# Autodesk Inventor assembly: intake part on end of six bar_MIR
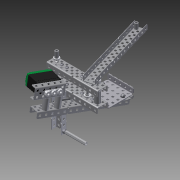
[picture p0: Inventor's stored thumbnail of the model, 180x180]
Saved by Autodesk Inventor 2014 SP1 (Build 180222100, 222)
## iProperties
Created: 2014-02-27
Part Number: intake part on end of six bar_MIR
Document SubType Name: Assembly
Designer: Ryan
Author: Ryan
## Documents named in this file (22)
- C:\Users\Ryan\Desktop\sw\toss up 4th robot\intake\intake part on end of six bar_MIR.iam
- C:\Users\Ryan\Desktop\sw\lib\Aperture VEX CAD Library\Metal\C Channel\2 x 10.ipt
- C:\Users\Ryan\Desktop\sw\lib\Aperture VEX CAD Library\Metal\C Channel\2 x 7.ipt
- C:\Users\Ryan\Desktop\sw\lib\Aperture VEX CAD Library\Bearing Blocks\Bearing Block.ipt
- C:\Users\Ryan\Desktop\sw\lib\Aperture VEX CAD Library\Metal\C Channel\5 x 5.ipt
- C:\Users\Ryan\Desktop\sw\lib\Aperture VEX CAD Library\Metal\vex hinge\hinge.iam
- C:\Users\Ryan\Desktop\sw\lib\Aperture VEX CAD Library\Spacers\SPACER-0500-0125.ipt
- C:\Users\Ryan\Desktop\sw\lib\Aperture VEX CAD Library\Spacers\SPACER-0500-0500.ipt
- C:\Users\Ryan\Desktop\sw\lib\Aperture VEX CAD Library\Spacers\SPACER-0500-0250.ipt
- C:\Users\Ryan\Desktop\sw\lib\Aperture VEX CAD Library\Metal\C Channel\2 x 15.ipt
- C:\Users\Ryan\Desktop\sw\toss up 4th robot\intake\4 hole long poly.ipt
- C:\Users\Ryan\Desktop\sw\lib\Aperture VEX CAD Library\Metal\C Channel\2 x 5.ipt
- C:\Users\Ryan\Desktop\sw\lib\Aperture VEX CAD Library\Motors\2-Wire Motor 393-Without Wire.iam
- C:\Users\Ryan\Desktop\sw\lib\Aperture VEX CAD Library\Standoffs\BEAM-2000.ipt
- C:\Users\Ryan\Desktop\sw\lib\Aperture VEX CAD Library\Hardware\8-32\8-32 nylock.ipt
- C:\Users\Ryan\Desktop\sw\lib\Aperture VEX CAD Library\Spacers\thin\SPACER-0320-0500.ipt
- C:\Users\Ryan\Desktop\sw\lib\Aperture VEX CAD Library\Hardware\8-32\8-32_.500.ipt
- C:\Users\Ryan\Desktop\sw\lib\Aperture VEX CAD Library\Hardware\8-32\8-32_.375.ipt
- C:\Users\Ryan\Desktop\sw\lib\Aperture VEX CAD Library\Hardware\8-32\8-32_.875.ipt
- C:\Users\Ryan\Desktop\sw\lib\Aperture VEX CAD Library\Hardware\8-32\8-32_1.750.ipt
- C:\Users\Ryan\Desktop\sw\lib\Aperture VEX CAD Library\Hardware\8-32\8-32 nylock_MIR7.ipt
- C:\Users\Ryan\Desktop\sw\lib\Aperture VEX CAD Library\Spacers\thin\SPACER-0320-00625.ipt
## Components (77 placed, 21 different names)
1. 2 x 10:1 — Flush:2, Flush:1, Flush:4, Flush:3, Mate:1, Mate:3, Mate:2, Mate:7, Mate:5, Mate:10, Mate:9, Mate:8, Mate:6, Flush:6, Flush:5, Mate:11, Mate:20, Mate:148
2. 2 x 10:2 — Flush:2, Flush:1, Mate:19, Mate:18, Mate:71, Mate:70, Mate:69, Mate:72, Mate:75, Mate:88, Mate:87, Mate:86, Mate:96, Mate:95, Mate:99, Mate:100, Mate:129, Mate:132, Mate:145, Mate:154
3. 2 x 7:1 — Flush:4, Flush:3, Mate:1, Mate:80, Mate:79, Mate:78
4. Bearing Block:1 — Mate:3, Mate:2, Mate:7, Mate:5, Mate:77, Mate:76, Mate:136
5. Bearing Block:2 — Mate:10, Mate:9, Mate:8, Mate:6, Mate:74, Mate:73, Mate:134
6. 5 x 5:1 — Flush:6, Flush:5, Mate:11, Flush:8, Flush:7, Mate:12, Mate:23, Mate:22, Mate:21, Mate:26, Mate:25, Mate:24, Mate:122, Mate:124
7. hinge:1 [sub-assembly] — Flush:8, Flush:7, Mate:12, Mate:29, Mate:28, Mate:27, Mate:126
8. SPACER-0500-0125:1 — Mate:15, Mate:16, Mate:146, Mate:147
9. SPACER-0500-0500:1 — Mate:20, Mate:15, Mate:14, Mate:13
10. SPACER-0500-0500:2 — Mate:19, Mate:18, Mate:16, Mate:14, Mate:13
11. SPACER-0500-0125:2 — Mate:23, Mate:22, Mate:21, Mate:118, Mate:117
12. SPACER-0500-0125:3 — Mate:26, Mate:25, Mate:24, Mate:120, Mate:119, Mate:121
13. SPACER-0500-0250:1 — Mate:29, Mate:28, Mate:27, Mate:30, Mate:35
14. 2 x 15:1 — Mate:30, Mate:33, Mate:32, Mate:31, Mate:40, Mate:39, Mate:38, Mate:37, Mate:36, Mate:46, Mate:45, Mate:44, Mate:53, Mate:52, Mate:51, Mate:110, Mate:112, Mate:142, Mate:144, Mate:139, Mate:141, Mate:142
15. Bearing Block:3 — Mate:35, Mate:33, Mate:32, Mate:31, Mate:109, Mate:111, Mate:114, Mate:115, Mate:125, Mate:128
16. SPACER-0500-0250:2 — Mate:40, Mate:39, Flush:9, Mate:43, Mate:137
17. SPACER-0500-0250:3 — Flush:9, Mate:38, Mate:37, Mate:36, Mate:42, Mate:41, Mate:139, Mate:141
18. 4 hole long poly:1 — Mate:43, Mate:42, Mate:41, Mate:138, Mate:140
19. SPACER-0500-0500:3 — Mate:46, Mate:45, Mate:44, Mate:48, Mate:47
20. SPACER-0500-0500:4 — Mate:48, Mate:47, Mate:57, Mate:54, Mate:140
21. SPACER-0500-0500:5 — Mate:53, Mate:52, Mate:51, Mate:50, Mate:49
22. SPACER-0500-0500:6 — Mate:50, Mate:49, Mate:56, Mate:55
23. 2 x 5:1 — Mate:57, Mate:56, Mate:55, Mate:54, Mate:61, Mate:60, Mate:59, Mate:58, Mate:62, Mate:140
24. Bearing Block:4 — Mate:61, Mate:60, Mate:59, Mate:58, Mate:64, Mate:63
25. 2-Wire Motor 393-Without Wire:1 [sub-assembly] — Mate:64, Mate:63, Mate:62
26. 2 x 15:2 — Mate:68, Mate:67, Mate:66, Mate:85, Mate:84, Mate:83
27. SPACER-0500-0125:4 — Mate:71, Mate:70, Mate:69, Mate:68, Mate:67, Mate:66, Mate:152, Mate:153
28. Bearing Block:5 — Mate:74, Mate:73, Mate:72, Mate:90, Mate:89, Mate:94, Mate:93, Mate:101, Mate:104, Mate:130
29. Bearing Block:6 — Mate:77, Mate:76, Mate:75, Mate:92, Mate:91, Mate:98, Mate:97, Mate:105, Mate:108, Mate:131
30. BEAM-2000:1 — Mate:82, Mate:81
31. 8-32 nylock:1 — Mate:82, Mate:81, Mate:80, Mate:79, Mate:78
32. SPACER-0320-0500:1 — Mate:85, Mate:84, Mate:83
33. SPACER-0320-0500:2 — Mate:88, Mate:87, Mate:86, Mate:155, Mate:156, Mate:157
34. SPACER-0500-0250:4 — Mate:90, Mate:89
35. SPACER-0500-0250:5 — Mate:92, Mate:91
36. 8-32_.500:5 — Mate:110, Mate:109, Mate:113
37. 8-32_.500:6 — Mate:112, Mate:111, Mate:116, Mate:139
38. 8-32 nylock:6 — Mate:114, Mate:113
39. 8-32 nylock:7 — Mate:116, Mate:115
40. 8-32_.375:1 — Mate:118, Mate:117, Mate:123
41. 8-32_.375:2 — Mate:120, Mate:119
42. 8-32 nylock:8 — Mate:122, Mate:121
43. 8-32 nylock:9 — Mate:124, Mate:123
44. 8-32_.875:1 — Mate:126, Mate:125, Mate:127
45. 8-32 nylock:10 — Mate:128, Mate:127
46. 8-32_1.750:1 — Mate:130, Mate:129, Mate:133
47. 8-32_1.750:2 — Mate:132, Mate:131, Mate:135, Mate:149, Mate:151
48. 8-32 nylock_MIR7:1 — Mate:134, Mate:133
49. 8-32 nylock:11 — Mate:136, Mate:135
50. 8-32_.500:7 — Mate:138, Mate:137, Mate:141
51. 8-32_.500:8 — Mate:140, Mate:139, Mate:143
52. 8-32 nylock:12 — Mate:142, Mate:141
53. 8-32 nylock:13 — Mate:144, Mate:143, Mate:142
54. SPACER-0500-0125:5 — Mate:143, Mate:144, Mate:146, Mate:147
55. SPACER-0500-0125:6 — Mate:143, Mate:144, Mate:145
56. SPACER-0500-0125:7 — Mate:148, Mate:149, Mate:150
57. SPACER-0320-00625:1 — Mate:150, Mate:151
58. SPACER-0500-0125:8 — Mate:152, Mate:153, Mate:158, Mate:159
59. SPACER-0500-0125:9 — Mate:154, Mate:155
60. SPACER-0320-00625:2 — Mate:156, Mate:157
61. SPACER-0320-00625:3 — Mate:158, Mate:159
62. 8-32_.500:3 — Mate:99, Mate:98, Mate:107
63. 8-32_.500:4 — Mate:100, Mate:97, Mate:106
64. 8-32_.500:1 — Mate:96, Mate:94, Mate:103
65. 8-32_.500:2 — Mate:95, Mate:93, Mate:102
66. 8-32 nylock:5 — Mate:108, Mate:107
67. 8-32 nylock:4 — Mate:106, Mate:105
68. 8-32 nylock:2 — Mate:102, Mate:101
69. 8-32 nylock:3 — Mate:104, Mate:103
70. 8-32_.500:9
71. 8-32_.500:10
72. 8-32_.500:11
73. 8-32_.500:12
74. 8-32 nylock:14
75. 8-32 nylock:15
76. 8-32 nylock:16
77. 8-32 nylock:17
## Component patterns: (2 elements, first: 8-32_.500:3 + 8-32_.500:4 + 8-32_.500:1 + 8-32_.500:2 + 8-32 nylock:5 + 8-32 nylock:4 + 8-32 nylock:2 + 8-32 nylock:3)
## Relationships (170: Mate 157, Flush 13)
- Flush:2: 2 x 10:1 ↔ 2 x 10:2
- Flush:1: 2 x 10:1 ↔ 2 x 10:2
- Flush:4: 2 x 10:1 ↔ 2 x 7:1
- Flush:3: 2 x 10:1 ↔ 2 x 7:1
- Mate:1: 2 x 10:1 ↔ 2 x 7:1
- Mate:3 (2.3114 mm): 2 x 10:1 ↔ Bearing Block:1
- Mate:2: 2 x 10:1 ↔ Bearing Block:1
- Mate:7 (2.3114 mm): 2 x 10:1 ↔ Bearing Block:1
- Mate:5 (2.3114 mm): 2 x 10:1 ↔ Bearing Block:1
- Mate:10 (2.3114 mm): 2 x 10:1 ↔ Bearing Block:2
- Mate:9 (2.3114 mm): 2 x 10:1 ↔ Bearing Block:2
- Mate:8 (2.3114 mm): 2 x 10:1 ↔ Bearing Block:2
- Mate:6: 2 x 10:1 ↔ Bearing Block:2
- Flush:6: 2 x 10:1 ↔ 5 x 5:1
- Flush:5: 2 x 10:1 ↔ 5 x 5:1
- Mate:11: 2 x 10:1 ↔ 5 x 5:1
- Flush:8: 5 x 5:1 ↔ hinge:1
- Flush:7: 5 x 5:1 ↔ hinge:1
- Mate:12: 5 x 5:1 ↔ hinge:1
- Mate:20: 2 x 10:1 ↔ SPACER-0500-0500:1
- Mate:15: SPACER-0500-0125:1 ↔ SPACER-0500-0500:1
- Mate:19 (2.3114 mm): 2 x 10:2 ↔ SPACER-0500-0500:2
- Mate:18 (2.3114 mm): 2 x 10:2 ↔ SPACER-0500-0500:2
- Mate:16: SPACER-0500-0125:1 ↔ SPACER-0500-0500:2
- Mate:14: SPACER-0500-0500:1 ↔ SPACER-0500-0500:2
- Mate:13: SPACER-0500-0500:1 ↔ SPACER-0500-0500:2
- Mate:23 (2.3114 mm): 5 x 5:1 ↔ SPACER-0500-0125:2
- Mate:22 (2.3114 mm): 5 x 5:1 ↔ SPACER-0500-0125:2
- Mate:21: 5 x 5:1 ↔ SPACER-0500-0125:2
- Mate:26 (2.3114 mm): 5 x 5:1 ↔ SPACER-0500-0125:3
- Mate:25 (2.3114 mm): 5 x 5:1 ↔ SPACER-0500-0125:3
- Mate:24: 5 x 5:1 ↔ SPACER-0500-0125:3
- Mate:29 (2.3114 mm): hinge:1 ↔ SPACER-0500-0250:1
- Mate:28 (2.3114 mm): hinge:1 ↔ SPACER-0500-0250:1
- Mate:27: hinge:1 ↔ SPACER-0500-0250:1
- Mate:30: SPACER-0500-0250:1 ↔ 2 x 15:1
- Mate:35: SPACER-0500-0250:1 ↔ Bearing Block:3
- Mate:33 (2.3114 mm): 2 x 15:1 ↔ Bearing Block:3
- Mate:32 (2.3114 mm): 2 x 15:1 ↔ Bearing Block:3
- Mate:31: 2 x 15:1 ↔ Bearing Block:3
- Mate:40 (2.3114 mm): 2 x 15:1 ↔ SPACER-0500-0250:2
- Mate:39 (2.3114 mm): 2 x 15:1 ↔ SPACER-0500-0250:2
- Flush:9: SPACER-0500-0250:2 ↔ SPACER-0500-0250:3
- Mate:38 (2.3114 mm): 2 x 15:1 ↔ SPACER-0500-0250:3
- Mate:37 (2.3114 mm): 2 x 15:1 ↔ SPACER-0500-0250:3
- Mate:36 [Flush]: 2 x 15:1 ↔ SPACER-0500-0250:3
- Mate:43: SPACER-0500-0250:2 ↔ 4 hole long poly:1
- Mate:42: SPACER-0500-0250:3 ↔ 4 hole long poly:1
- Mate:41: SPACER-0500-0250:3 ↔ 4 hole long poly:1
- Mate:46 (2.3114 mm): 2 x 15:1 ↔ SPACER-0500-0500:3
- Mate:45: 2 x 15:1 ↔ SPACER-0500-0500:3
- Mate:44 (-10.3886 mm): 2 x 15:1 ↔ SPACER-0500-0500:3
- Mate:48: SPACER-0500-0500:3 ↔ SPACER-0500-0500:4
- Mate:47: SPACER-0500-0500:3 ↔ SPACER-0500-0500:4
- Mate:53 (2.3114 mm): 2 x 15:1 ↔ SPACER-0500-0500:5
- Mate:52 (-10.3886 mm): 2 x 15:1 ↔ SPACER-0500-0500:5
- Mate:51: 2 x 15:1 ↔ SPACER-0500-0500:5
- Mate:50: SPACER-0500-0500:5 ↔ SPACER-0500-0500:6
- Mate:49: SPACER-0500-0500:5 ↔ SPACER-0500-0500:6
- Mate:57 (2.3114 mm): SPACER-0500-0500:4 ↔ 2 x 5:1
- Mate:56 (2.3114 mm): SPACER-0500-0500:6 ↔ 2 x 5:1
- Mate:55 (2.3114 mm): SPACER-0500-0500:6 ↔ 2 x 5:1
- Mate:54 [Flush]: SPACER-0500-0500:4 ↔ 2 x 5:1
- Mate:61 (2.3114 mm): 2 x 5:1 ↔ Bearing Block:4
- Mate:60 (2.3114 mm): 2 x 5:1 ↔ Bearing Block:4
- Mate:59 (2.3114 mm): 2 x 5:1 ↔ Bearing Block:4
- Mate:58: 2 x 5:1 ↔ Bearing Block:4
- Mate:64: Bearing Block:4 ↔ 2-Wire Motor 393-Without Wire:1
- Mate:63: Bearing Block:4 ↔ 2-Wire Motor 393-Without Wire:1
- Mate:62: 2 x 5:1 ↔ 2-Wire Motor 393-Without Wire:1
- Mate:71 (2.3114 mm): 2 x 10:2 ↔ SPACER-0500-0125:4
- Mate:70 (2.3114 mm): 2 x 10:2 ↔ SPACER-0500-0125:4
- Mate:69: 2 x 10:2 ↔ SPACER-0500-0125:4
- Mate:68 (4.7625 mm): 2 x 15:2 ↔ SPACER-0500-0125:4
- Mate:67 (2.3114 mm): 2 x 15:2 ↔ SPACER-0500-0125:4
- Mate:66 (2.3114 mm): 2 x 15:2 ↔ SPACER-0500-0125:4
- Mate:74: Bearing Block:2 ↔ Bearing Block:5
- Mate:73: Bearing Block:2 ↔ Bearing Block:5
- Mate:72: 2 x 10:2 ↔ Bearing Block:5
- Mate:77: Bearing Block:1 ↔ Bearing Block:6
- Mate:76: Bearing Block:1 ↔ Bearing Block:6
- Mate:75: 2 x 10:2 ↔ Bearing Block:6
- Mate:82: BEAM-2000:1 ↔ 8-32 nylock:1
- Mate:81: BEAM-2000:1 ↔ 8-32 nylock:1
- Mate:80 (2.3114 mm): 2 x 7:1 ↔ 8-32 nylock:1
- Mate:79 (2.3114 mm): 2 x 7:1 ↔ 8-32 nylock:1
- Mate:78: 2 x 7:1 ↔ 8-32 nylock:1
- Mate:85 (2.3114 mm): 2 x 15:2 ↔ SPACER-0320-0500:1
- Mate:84: 2 x 15:2 ↔ SPACER-0320-0500:1
- Mate:83 (2.3114 mm): 2 x 15:2 ↔ SPACER-0320-0500:1
- Mate:88 (2.3114 mm): 2 x 10:2 ↔ SPACER-0320-0500:2
- Mate:87 (2.3114 mm): 2 x 10:2 ↔ SPACER-0320-0500:2
- Mate:86 (3.175 mm): 2 x 10:2 ↔ SPACER-0320-0500:2
- Mate:90: Bearing Block:5 ↔ SPACER-0500-0250:4
- Mate:89: Bearing Block:5 ↔ SPACER-0500-0250:4
- Mate:92: Bearing Block:6 ↔ SPACER-0500-0250:5
- Mate:91: Bearing Block:6 ↔ SPACER-0500-0250:5
- Mate:96: 2 x 10:2 ↔ 8-32_.500:1
- Mate:94: Bearing Block:5 ↔ 8-32_.500:1
- Mate:95: 2 x 10:2 ↔ 8-32_.500:2
- Mate:93: Bearing Block:5 ↔ 8-32_.500:2
- Mate:99: 2 x 10:2 ↔ 8-32_.500:3
- Mate:98: Bearing Block:6 ↔ 8-32_.500:3
- Mate:100: 2 x 10:2 ↔ 8-32_.500:4
- Mate:97: Bearing Block:6 ↔ 8-32_.500:4
- Mate:102: 8-32_.500:2 ↔ 8-32 nylock:2
- Mate:101: Bearing Block:5 ↔ 8-32 nylock:2
- Mate:104: Bearing Block:5 ↔ 8-32 nylock:3
- Mate:103: 8-32_.500:1 ↔ 8-32 nylock:3
- Mate:106: 8-32_.500:4 ↔ 8-32 nylock:4
- Mate:105: Bearing Block:6 ↔ 8-32 nylock:4
- Mate:108: Bearing Block:6 ↔ 8-32 nylock:5
- Mate:107: 8-32_.500:3 ↔ 8-32 nylock:5
- Mate:110: 2 x 15:1 ↔ 8-32_.500:5
- Mate:109: Bearing Block:3 ↔ 8-32_.500:5
- Mate:112: 2 x 15:1 ↔ 8-32_.500:6
- Mate:111: Bearing Block:3 ↔ 8-32_.500:6
- Mate:114: Bearing Block:3 ↔ 8-32 nylock:6
- Mate:113: 8-32_.500:5 ↔ 8-32 nylock:6
- Mate:116: 8-32_.500:6 ↔ 8-32 nylock:7
- Mate:115: Bearing Block:3 ↔ 8-32 nylock:7
- Mate:118: SPACER-0500-0125:2 ↔ 8-32_.375:1
- Mate:117: SPACER-0500-0125:2 ↔ 8-32_.375:1
- Mate:120: SPACER-0500-0125:3 ↔ 8-32_.375:2
- Mate:119: SPACER-0500-0125:3 ↔ 8-32_.375:2
- Mate:122: 5 x 5:1 ↔ 8-32 nylock:8
- Mate:121: SPACER-0500-0125:3 ↔ 8-32 nylock:8
- Mate:124: 5 x 5:1 ↔ 8-32 nylock:9
- Mate:123: 8-32_.375:1 ↔ 8-32 nylock:9
- Mate:126: hinge:1 ↔ 8-32_.875:1
- Mate:125: Bearing Block:3 ↔ 8-32_.875:1
- Mate:128: Bearing Block:3 ↔ 8-32 nylock:10
- Mate:127: 8-32_.875:1 ↔ 8-32 nylock:10
- Mate:130: Bearing Block:5 ↔ 8-32_1.750:1
- Mate:129: 2 x 10:2 ↔ 8-32_1.750:1
- Mate:132: 2 x 10:2 ↔ 8-32_1.750:2
- Mate:131: Bearing Block:6 ↔ 8-32_1.750:2
- Mate:134: Bearing Block:2 ↔ 8-32 nylock_MIR7:1
- Mate:133: 8-32_1.750:1 ↔ 8-32 nylock_MIR7:1
- Mate:136: Bearing Block:1 ↔ 8-32 nylock:11
- Mate:135: 8-32_1.750:2 ↔ 8-32 nylock:11
- Mate:138: 4 hole long poly:1 ↔ 8-32_.500:7
- Mate:137: SPACER-0500-0250:2 ↔ 8-32_.500:7
- Mate:140: 4 hole long poly:1 ↔ 8-32_.500:8
- Mate:139: SPACER-0500-0250:3 ↔ 8-32_.500:8
- Mate:142 [Flush]: 2 x 15:1 ↔ 8-32 nylock:12
- Mate:141: 8-32_.500:7 ↔ 8-32 nylock:12
- Mate:144 [Flush]: 2 x 15:1 ↔ 8-32 nylock:13
- Mate:143: 8-32_.500:8 ↔ 8-32 nylock:13
- Mate:139 (2.3114 mm): 2 x 15:1 ↔ 8-32_.500:6
- Mate:140: SPACER-0500-0500:4 ↔ 2 x 5:1
- Mate:141: 2 x 15:1 ↔ SPACER-0500-0250:3
- Mate:142: 2 x 15:1 ↔ 8-32 nylock:13
- Mate:143: SPACER-0500-0125:5 ↔ SPACER-0500-0125:6
- Mate:144: SPACER-0500-0125:5 ↔ SPACER-0500-0125:6
- Mate:145: 2 x 10:2 ↔ SPACER-0500-0125:6
- Mate:146: SPACER-0500-0125:1 ↔ SPACER-0500-0125:5
- Mate:147: SPACER-0500-0125:1 ↔ SPACER-0500-0125:5
- Mate:148: 2 x 10:1 ↔ SPACER-0500-0125:7
- Mate:149: 8-32_1.750:2 ↔ SPACER-0500-0125:7
- Mate:150: SPACER-0500-0125:7 ↔ SPACER-0320-00625:1
- Mate:151: 8-32_1.750:2 ↔ SPACER-0320-00625:1
- Mate:152: SPACER-0500-0125:4 ↔ SPACER-0500-0125:8
- Mate:153: SPACER-0500-0125:4 ↔ SPACER-0500-0125:8
- Mate:154: 2 x 10:2 ↔ SPACER-0500-0125:9
- Mate:155: SPACER-0320-0500:2 ↔ SPACER-0500-0125:9
- Mate:156: SPACER-0320-0500:2 ↔ SPACER-0320-00625:2
- Mate:157: SPACER-0320-0500:2 ↔ SPACER-0320-00625:2
- Mate:158: SPACER-0500-0125:8 ↔ SPACER-0320-00625:3
- Mate:159: SPACER-0500-0125:8 ↔ SPACER-0320-00625:3
